# Autodesk Inventor assembly: jorneFester
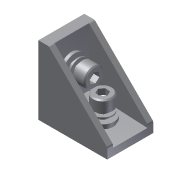
[picture p0: Inventor's stored thumbnail of the model, 180x180]
Saved by Autodesk Inventor 2014 SP1 (Build 180222100, 222)
## iProperties
Created: 2015-02-04
Part Number: jorneFester
Document SubType Name: Assembly
Designer: Simen
Author: Simen
## Documents named in this file (3)
- C:\Users\Simen\Documents\git\Eit\skjellet\jorneFester.iam
- C:\Users\Simen\Documents\git\Eit\skjellet\mutterOgSkrue.iam
- C:\Users\Simen\Documents\git\Eit\skjellet\HBLFSN5.iam
## Components (3 placed, 2 different names)
1. mutterOgSkrue:2 [sub-assembly] — Mate:1, Mate:2
2. HBLFSN5:1 [sub-assembly] — Mate:1, Mate:2, Mate:3, Mate:4
3. mutterOgSkrue:3 [sub-assembly] — Mate:3, Mate:4
## Relationships (4: Mate 4)
- Mate:1: mutterOgSkrue:2 ↔ HBLFSN5:1
- Mate:2: mutterOgSkrue:2 ↔ HBLFSN5:1
- Mate:3: HBLFSN5:1 ↔ mutterOgSkrue:3
- Mate:4: HBLFSN5:1 ↔ mutterOgSkrue:3
